# Autodesk Inventor assembly: Manette
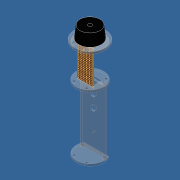
[picture p0: Inventor's stored thumbnail of the model, 180x180]
Saved by Autodesk Inventor 2015 SP2 (Build 190223200, 223)
## iProperties
Created: 2018-03-23
Part Number: Manette
Project: Nom Projet
Description: Ens. Nom Ensemble
Document SubType Name: Assembly
Designer: Alexandre.PICOTTE
Author: Alexandre.PICOTTE
## Documents named in this file (9)
- C:\Users\Alexandre.PICOTTE\Documents\P1704_Manette\06_Dessins\Concept de souris\Manette.iam
- C:\Users\Alexandre.PICOTTE\Documents\P1704_Manette\06_Dessins\Concept de souris\Couvercle_bas.ipt
- C:\Users\Alexandre.PICOTTE\Documents\P1704_Manette\06_Dessins\Concept de souris\Paroi_interne.ipt
- C:\Users\Alexandre.PICOTTE\Documents\P1704_Manette\06_Dessins\Concept de souris\Couvercle_replat.ipt
- C:\Users\Alexandre.PICOTTE\Documents\P1704_Manette\06_Dessins\Concept de souris\Couvercle_haut.ipt
- C:\Users\Alexandre.PICOTTE\Documents\P1704_Manette\06_Dessins\Concept de souris\Couvercle_rail.ipt
- C:\Users\Alexandre.PICOTTE\Documents\P1704_Manette\06_Dessins\Concept de souris\Encodeur.ipt
- C:\Users\Alexandre.PICOTTE\Documents\P1704_Manette\06_Dessins\Concept de souris\Veroboard.ipt
- C:\Users\Alexandre.PICOTTE\Documents\P1704_Manette\06_Dessins\Concept de souris\Molette.ipt
## Components (8 placed, 8 different names)
1. Couvercle_bas:1 — Placage:20, Placage:21, Placage:22
2. Couvercle_replat:1 — Placage:9, Placage:13, Placage:17, Placage:18, Placage:19, Placage:25
3. Couvercle_haut:1 — Placage:6, Placage:7, Placage:8, Placage:9, Placage:10, Placage:11, Placage:12, Placage:13, Placage:16, Placage:24
4. Couvercle_rail:1 — Placage:6, Placage:7, Placage:8, Placage:14, Placage:15, Placage:25
5. Encodeur:1 — Placage:10, Placage:11, Placage:12, Placage:23
6. Veroboard:1 — Placage:14, Placage:15, Placage:16
7. Paroi_interne:1 — Placage:17, Placage:18, Placage:19, Placage:20, Placage:21, Placage:22
8. Molette:1 — Placage:23, Placage:24
## Relationships (20: Mate 20)
- Placage:6 [Mate]: Couvercle_haut:1 ↔ Couvercle_rail:1
- Placage:7 [Mate]: Couvercle_haut:1 ↔ Couvercle_rail:1
- Placage:8 [Mate]: Couvercle_haut:1 ↔ Couvercle_rail:1
- Placage:9 [Mate]: Couvercle_replat:1 ↔ Couvercle_haut:1
- Placage:10 [Mate]: Couvercle_haut:1 ↔ Encodeur:1
- Placage:11 [Mate]: Couvercle_haut:1 ↔ Encodeur:1
- Placage:12 [Mate]: Couvercle_haut:1 ↔ Encodeur:1
- Placage:13 [Mate]: Couvercle_replat:1 ↔ Couvercle_haut:1
- Placage:14 [Mate]: Couvercle_rail:1 ↔ Veroboard:1
- Placage:15 [Mate]: Couvercle_rail:1 ↔ Veroboard:1
- Placage:16 [Mate]: Couvercle_haut:1 ↔ Veroboard:1
- Placage:17 [Mate]: Couvercle_replat:1 ↔ Paroi_interne:1
- Placage:18 [Mate]: Couvercle_replat:1 ↔ Paroi_interne:1
- Placage:19 [Mate]: Couvercle_replat:1 ↔ Paroi_interne:1
- Placage:20 [Mate]: Couvercle_bas:1 ↔ Paroi_interne:1
- Placage:21 [Mate]: Couvercle_bas:1 ↔ Paroi_interne:1
- Placage:22 [Mate]: Couvercle_bas:1 ↔ Paroi_interne:1
- Placage:23 [Mate]: Encodeur:1 ↔ Molette:1
- Placage:24 [Mate] (1 mm): Couvercle_haut:1 ↔ Molette:1
- Placage:25 [Mate] (50 mm): Couvercle_replat:1 ↔ Couvercle_rail:1
